# Autodesk Inventor assembly: Motor Assembly
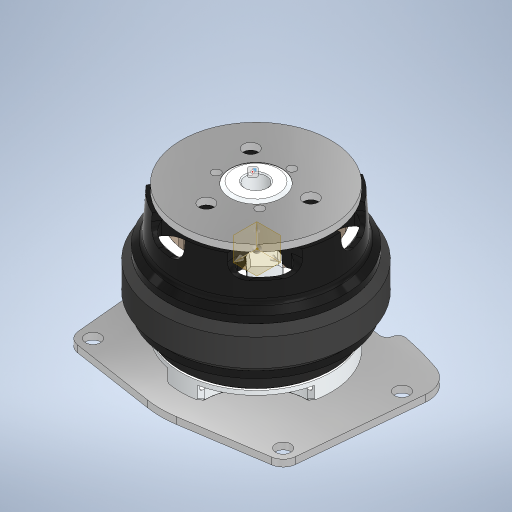
[picture p0: Inventor's stored thumbnail of the model, 512x512]
Saved by Autodesk Inventor 2023.2 (Build 272271000, 271)
## iProperties
Created: 2022-12-29
Part Number: Motor Assembly
Document SubType Name: Assembly
Designer: Nathan Cai
Mass: 22.5339 g
Surface Area: 305.453 cm^2
Volume: 18.6872 cm^3
Density: 1.20585 g/cm^3
Author: Nathan Cai
## Documents named in this file (6)
- E:\Documents\Inventor\Moon Cake V0.13\Motor Assembly.iam
- E:\Documents\Inventor\Moon Cake V0.13\Propdrive 3536\Propdrive V2 3536.iam
- E:\Documents\Inventor\Moon Cake V0.13\Motor Cap.ipt
- E:\Documents\Inventor\Moon Cake V0.13\Motor Hub.ipt
- E:\Documents\Inventor\Moon Cake V0.13\Motor Clutch.ipt
- E:\Documents\Inventor\Moon Cake V0.13\Motor Plate.ipt
## Components (5 placed, 5 different names)
1. Propdrive V2 3536:1 [sub-assembly] — Mate:1, Mate:2, Mate:3, Mate:4, Mate:9, Mate:10, Mate:11
2. Motor Cap:1 — Mate:1, Mate:2, Mate:3, Mate:7, Mate:8
3. Motor Hub:1 — Mate:4, Mate:5, Mate:6, Mate:7, Mate:8
4. Motor Clutch:1 — Mate:5, Mate:6
5. Motor Plate:1 — Mate:9, Mate:10, Mate:11
## Relationships (11: Mate 11)
- Mate:1: Propdrive V2 3536:1 ↔ Motor Cap:1
- Mate:2: Propdrive V2 3536:1 ↔ Motor Cap:1
- Mate:3: Propdrive V2 3536:1 ↔ Motor Cap:1
- Mate:4: Propdrive V2 3536:1 ↔ Motor Hub:1
- Mate:5: Motor Hub:1 ↔ Motor Clutch:1
- Mate:6: Motor Hub:1 ↔ Motor Clutch:1
- Mate:7: Motor Cap:1 ↔ Motor Hub:1
- Mate:8: Motor Cap:1 ↔ Motor Hub:1
- Mate:9: Propdrive V2 3536:1 ↔ Motor Plate:1
- Mate:10: Propdrive V2 3536:1 ↔ Motor Plate:1
- Mate:11: Propdrive V2 3536:1 ↔ Motor Plate:1
